# Autodesk Inventor assembly: Cube 1x1 V5
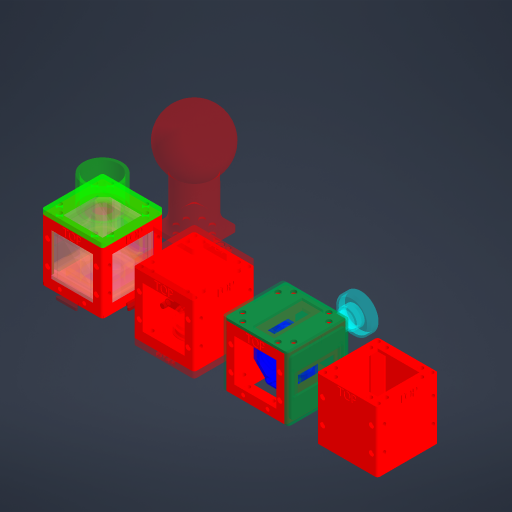
[picture p0: Inventor's stored thumbnail of the model, 512x512]
Saved by Autodesk Inventor 2023.4 (Build 274418000, 418)
## iProperties
Created: 2022-07-25
Part Number: Cube 1x1 V5
Document SubType Name: Assembly
Designer: xSibe
Author: xSibe
## Documents named in this file (60)
- C:\.Laptop\.Work\Projects\Project Protocube\Protocube\CAD, STL, OBJ Files\1 CAD\Cube 1x1 V5.iam
- C:\.Laptop\.Work\Projects\Project Protocube\Protocube\CAD, STL, OBJ Files\1 CAD\Cubes\Cube 1x1 Bottom V5.ipt
- C:\.Laptop\.Work\Projects\Project Protocube\Protocube\CAD, STL, OBJ Files\1 CAD\Cubes\Cube 1x1 Top V5.ipt
- C:\.Laptop\.Work\Projects\Project Protocube\Protocube\CAD, STL, OBJ Files\1 CAD\Lens\One Inch Lens Mount (V5).ipt
- C:\.Laptop\.Work\Projects\Project Protocube\Protocube\CAD, STL, OBJ Files\1 CAD\Lens\Half Inch Lens Mount (V5).ipt
- C:\.Laptop\.Work\Projects\Project Protocube\Protocube\CAD, STL, OBJ Files\1 CAD\Objective\Objective Mount.ipt
- C:\.Laptop\.Work\Projects\Project Protocube\Protocube\CAD, STL, OBJ Files\1 CAD\Mirror\Mirror Base Vertical.ipt
- C:\.Laptop\.Work\Projects\Project Protocube\Protocube\CAD, STL, OBJ Files\1 CAD\Mirror\Mirror Plate Vertical.ipt
- C:\.Laptop\.Work\Projects\Project Protocube\Protocube\CAD, STL, OBJ Files\1 CAD\Dichroic\Dichroic Mirror Mount.ipt
- C:\.Laptop\.Work\Projects\Project Protocube\Protocube\CAD, STL, OBJ Files\1 CAD\Accessories\Top Mount (SM1).ipt
- C:\.Laptop\.Work\Projects\Project Protocube\Protocube\CAD, STL, OBJ Files\1 CAD\Accessories\Flashlight Mount V1.ipt
- C:\.Laptop\.Work\Projects\Project Protocube\Protocube\CAD, STL, OBJ Files\1 CAD\Camera\Camera Mount Side.ipt
- C:\.Laptop\.Work\Projects\Project Protocube\Protocube\CAD, STL, OBJ Files\1 CAD\Lens\SM1 Lens Mount (V5).ipt
- C:\.Laptop\.Work\Projects\Project Protocube\Protocube\CAD, STL, OBJ Files\1 CAD\Mirror\Mirror Base Horizontal.ipt
- C:\.Laptop\.Work\Projects\Project Protocube\Protocube\CAD, STL, OBJ Files\1 CAD\Mirror\Mirror Plate Horizontal.ipt
- C:\.Laptop\.Work\Projects\Project Protocube\Protocube\CAD, STL, OBJ Files\1 CAD\Tools\Baseplate V5 Press.ipt
- C:\.Laptop\.Work\Projects\Project Protocube\Protocube\CAD, STL, OBJ Files\1 CAD\Tools\Laser Alignment Tool V1.ipt
- C:\.Laptop\.Work\Projects\Project Protocube\Protocube\CAD, STL, OBJ Files\1 CAD\Filter\Filter Mount (SM05).ipt
- C:\.Laptop\.Work\Projects\Project Protocube\Protocube\CAD, STL, OBJ Files\1 CAD\Filter\Filter Mount (SM1).ipt
- C:\.Laptop\.Work\Projects\Project Protocube\Protocube\CAD, STL, OBJ Files\1 CAD\Covers\Inner Cover Side.ipt
- C:\.Laptop\.Work\Projects\Project Protocube\Protocube\CAD, STL, OBJ Files\1 CAD\Covers\Inner Cover Side Open.ipt
- C:\.Laptop\.Work\Projects\Project Protocube\Protocube\CAD, STL, OBJ Files\1 CAD\Cubes\Cube 1x1 Top V5 Closed.ipt
- C:\.Laptop\.Work\Projects\Project Protocube\Protocube\CAD, STL, OBJ Files\1 CAD\Cubes\Cube 1x1 Bottom V5 Closed.ipt
- C:\.Laptop\.Work\Projects\Project Protocube\Protocube\CAD, STL, OBJ Files\1 CAD\Cubes\Cube 1x1 Bottom V5 Closed Slotted.ipt
- C:\.Laptop\.Work\Projects\Project Protocube\Protocube\CAD, STL, OBJ Files\1 CAD\Cubes\Cube 1x1 Top V5 Closed Slotted.ipt
- C:\.Laptop\.Work\Projects\Project Protocube\Protocube\CAD, STL, OBJ Files\1 CAD\Lens\Half Inch Lens Mount Cover (V5).ipt
- C:\.Laptop\.Work\Projects\Project Protocube\Protocube\CAD, STL, OBJ Files\1 CAD\Lens\One Inch Lens Mount Cover (V5).ipt
- C:\.Laptop\.Work\Projects\Project Protocube\Protocube\CAD, STL, OBJ Files\1 CAD\Tools\Laser Alignment Tool V2.ipt
- C:\.Laptop\.Work\Projects\Project Protocube\Protocube\CAD, STL, OBJ Files\1 CAD\Lens\SM05 Lens Mount (V5).ipt
- C:\.Laptop\.Work\Projects\Project Protocube\Protocube\CAD, STL, OBJ Files\1 CAD\Laser\Laser Switch.ipt
- C:\.Laptop\.Work\Projects\Project Protocube\Protocube\CAD, STL, OBJ Files\1 CAD\Laser\Laser Holder (USB Laser).ipt
- C:\.Laptop\.Work\Projects\Project Protocube\Protocube\CAD, STL, OBJ Files\1 CAD\XYZ Stage\Z Stage Body V5.ipt
- C:\.Laptop\.Work\Projects\Project Protocube\Protocube\CAD, STL, OBJ Files\1 CAD\Accessories\Top Mount (SM05).ipt
- C:\.Laptop\.Work\Projects\Project Protocube\Protocube\CAD, STL, OBJ Files\1 CAD\Tools\Cube 1x1 V5 Bot Press.ipt
- C:\.Laptop\.Work\Projects\Project Protocube\Protocube\CAD, STL, OBJ Files\1 CAD\Tools\Cube 1x1 V5 Top Press.ipt
- C:\.Laptop\.Work\Projects\Project Protocube\Protocube\CAD, STL, OBJ Files\1 CAD\Filter\Filter Adapter (SM1).ipt
- C:\.Laptop\.Work\Projects\Project Protocube\Protocube\CAD, STL, OBJ Files\1 CAD\Filter\Filter Adapter (SM05).ipt
- C:\.Laptop\.Work\Projects\Project Protocube\Protocube\CAD, STL, OBJ Files\1 CAD\Laser\Laser Holder (Smaller).ipt
- C:\.Laptop\.Work\Projects\Project Protocube\Protocube\CAD, STL, OBJ Files\1 CAD\Cubes\Cube 1x1 Bottom V5 Closed Vertical.ipt
- C:\.Laptop\.Work\Projects\Project Protocube\Protocube\CAD, STL, OBJ Files\1 CAD\Sample\Sample Holder.ipt
- C:\.Laptop\.Work\Projects\Project Protocube\Protocube\CAD, STL, OBJ Files\1 CAD\Sample\Sample Clamp.ipt
- C:\.Laptop\.Work\Projects\Project Protocube\Protocube\CAD, STL, OBJ Files\1 CAD\Tools\SM1 Press Inner.ipt
- C:\.Laptop\.Work\Projects\Project Protocube\Protocube\CAD, STL, OBJ Files\1 CAD\Tools\SM1 Press Outer.ipt
- C:\.Laptop\.Work\Projects\Project Protocube\Protocube\CAD, STL, OBJ Files\1 CAD\Covers\Outer Cover Open.ipt
- C:\.Laptop\.Work\Projects\Project Protocube\Protocube\CAD, STL, OBJ Files\1 CAD\Baseplates\Interlinking Baseplate.ipt
- C:\.Laptop\.Work\Projects\Project Protocube\Protocube\CAD, STL, OBJ Files\1 CAD\Accessories\Tunnel Vertical.ipt
- C:\.Laptop\.Work\Projects\Project Protocube\Protocube\CAD, STL, OBJ Files\1 CAD\Accessories\Tunnel Horizontal.ipt
- C:\.Laptop\.Work\Projects\Project Protocube\Protocube\CAD, STL, OBJ Files\1 CAD\Baseplates\Interlinking Baseplate Spacer.ipt
- C:\.Laptop\.Work\Projects\Project Protocube\Protocube\CAD, STL, OBJ Files\1 CAD\Baseplates\Interlinking Baseplate Pathed.ipt
- C:\.Laptop\.Work\Projects\Project Protocube\Protocube\CAD, STL, OBJ Files\1 CAD\Baseplates\Interlinking Baseplate Pathed Male.ipt
- C:\.Laptop\.Work\Projects\Project Protocube\Protocube\CAD, STL, OBJ Files\1 CAD\Baseplates\Interlinking Baseplate Pathed Female.ipt
- C:\.Laptop\.Work\Projects\Project Protocube\Protocube\CAD, STL, OBJ Files\1 CAD\Baseplates\Interlinking Baseplate Pathed Angle V2.ipt
- C:\.Laptop\.Work\Projects\Project Protocube\Protocube\CAD, STL, OBJ Files\1 CAD\Baseplates\Interlinking Baseplate Pathed Angle V1.ipt
- C:\.Laptop\.Work\Projects\Project Protocube\Protocube\CAD, STL, OBJ Files\1 CAD\Covers\Outer Cover Top Open.ipt
- C:\.Laptop\.Work\Projects\Project Protocube\Protocube\CAD, STL, OBJ Files\1 CAD\Tools\SM1 Removal Tool.ipt
- C:\.Laptop\.Work\Projects\Project Protocube\Protocube\CAD, STL, OBJ Files\1 CAD\Covers\Outer Cover.ipt
- C:\.Laptop\.Work\Projects\Project Protocube\Protocube\CAD, STL, OBJ Files\1 CAD\Covers\Outer Cover Top.ipt
- C:\.Laptop\.Work\Projects\Project Protocube\Protocube\CAD, STL, OBJ Files\1 CAD\Covers\Outer Cover Full.ipt
- C:\.Laptop\.Work\Projects\Project Protocube\Protocube\CAD, STL, OBJ Files\1 CAD\Covers\Outer Cover Side Open.ipt
- C:\.Laptop\.Work\Projects\Project Protocube\Protocube\CAD, STL, OBJ Files\1 CAD\Covers\Outer Cover Side.ipt
## Components (60 placed, 59 different names)
1. Cube 1x1 Top V5:1 — Mate:1, Mate:2, Mate:3, Mate:4, Mate:5, Mate:6, Mate:40, Flush:23, Flush:24, Mate:60, Mate:61, Mate:62, Mate:63, Mate:64, Mate:65, Flush:39
2. Cube 1x1 Bottom V5:1 — Mate:1, Mate:2, Mate:3, Mate:39, Flush:21, Mate:70, Mate:85, Flush:35, Flush:36, Mate:86, Flush:37
3. Cube 1x1 Top V5 Closed:1 — Mate:40, Flush:23, Flush:24, Mate:41, Mate:42, Mate:43, Mate:77, Mate:78, Mate:79
4. Cube 1x1 Bottom V5 Closed:1 — Mate:41, Mate:42, Mate:43, Mate:54, Mate:55, Mate:56, Mate:76, Mate:80, Mate:81, Mate:82, Mate:83, Flush:30, Mate:75
5. Cube 1x1 Top V5 Closed Slotted:1 — Mate:51, Mate:52, Mate:53
6. Cube 1x1 Bottom V5 Closed Slotted:1 — Mate:51, Mate:52, Mate:53, Mate:54, Mate:55, Mate:56, Mate:66, Flush:25, Flush:26, Flush:32, Flush:33, Flush:34, Flush:42
7. Cube 1x1 Top V5:2 — Mate:67, Mate:68, Mate:69
8. Cube 1x1 Bottom V5 Closed Vertical:1 — Mate:66, Flush:25, Flush:26, Mate:67, Mate:68, Mate:69
9. Laser Alignment Tool V1:1 — Flush:18
10. Laser Alignment Tool V2:1
11. Baseplate V5 Press:1 — Flush:15
12. Cube 1x1 V5 Bot Press:1 — Mate:76, Mate:80, Mate:81
13. Cube 1x1 V5 Top Press:1 — Mate:77, Mate:78, Mate:79
14. SM1 Removal Tool:1 — Mate:87, Flush:40, Flush:41
15. SM1 Press Outer:1 — Flush:29, Mate:74, Mate:75, Flush:40, Flush:41
16. SM1 Press Inner:1 — Flush:29, Mate:74, Mate:87
17. Laser Switch:1 — Mate:82, Mate:83, Flush:30
18. Z Stage Body V5:1
19. Half Inch Lens Mount Cover (V5):1
20. One Inch Lens Mount Cover (V5):1
21. Half Inch Lens Mount (V5):1
22. One Inch Lens Mount (V5):1 — Flush:1
23. SM05 Lens Mount (V5):1
24. SM1 Lens Mount (V5):1
25. Filter Mount (SM05):1 — Flush:19
26. Filter Mount (SM1):1
27. Laser Holder (USB Laser):1
28. Laser Holder (Smaller):1
29. Mirror Base Vertical:1 — Flush:5
30. Mirror Plate Vertical:1
31. Mirror Base Horizontal:1 — Flush:12, Flush:14
32. Mirror Plate Horizontal:1 — Mate:38, Flush:13, Flush:14
33. Dichroic Mirror Mount:1 — Flush:6
34. Camera Mount Side:1 — Flush:7
35. Objective Mount:1 — Flush:4
36. Tunnel Horizontal:1 — Mate:86, Flush:37, Flush:39
37. Tunnel Vertical:1 — Mate:85, Flush:35, Flush:36
38. Sample Holder:1 — Mate:70, Mate:71, Flush:27, Mate:72
39. Sample Clamp:1 — Mate:72, Mate:73, Flush:28
40. Interlinking Baseplate:1
41. Interlinking Baseplate Spacer:1
42. Interlinking Baseplate Pathed:1
43. Interlinking Baseplate Pathed Male:1
44. Interlinking Baseplate Pathed Female:1
45. Interlinking Baseplate Pathed Angle V2:1
46. Interlinking Baseplate Pathed Angle V1:1
47. Filter Adapter (SM1):1 — Mate:84, Flush:31, Flush:32, Flush:33, Flush:34
48. Filter Adapter (SM05):1 — Mate:84, Flush:31
49. Top Mount (SM1):1 — Mate:4, Mate:5, Mate:6
50. Top Mount (SM05):1 — Mate:60, Mate:61, Mate:62
51. Flashlight Mount V1:1 — Mate:63, Mate:64, Mate:65
52. Outer Cover Side Open:1 — Flush:42, Flush:43
53. Outer Cover Side:1 — Flush:43
54. Outer Cover Top Open:1
55. Outer Cover Top:1
56. Outer Cover Open:1
57. Outer Cover:1
58. Outer Cover Full:1
59. Inner Cover Side:1 — Flush:20, Mate:39, Flush:21
60. Inner Cover Side Open:1
## Relationships (79: Mate 46, Flush 33)
- Mate:1: Cube 1x1 Top V5:1 ↔ Cube 1x1 Bottom V5:1
- Mate:2: Cube 1x1 Top V5:1 ↔ Cube 1x1 Bottom V5:1
- Mate:3: Cube 1x1 Top V5:1 ↔ Cube 1x1 Bottom V5:1
- Flush:1: One Inch Lens Mount (V5):1
- Flush:4: Objective Mount:1
- Flush:5: Mirror Base Vertical:1
- Flush:6: Dichroic Mirror Mount:1
- Mate:4: Cube 1x1 Top V5:1 ↔ Top Mount (SM1):1
- Mate:5: Cube 1x1 Top V5:1 ↔ Top Mount (SM1):1
- Mate:6: Cube 1x1 Top V5:1 ↔ Top Mount (SM1):1
- Flush:7: Camera Mount Side:1
- Flush:12: Mirror Base Horizontal:1
- Mate:38: Mirror Plate Horizontal:1
- Flush:13: Mirror Plate Horizontal:1
- Flush:14: Mirror Base Horizontal:1 ↔ Mirror Plate Horizontal:1
- Flush:15: Baseplate V5 Press:1
- Flush:18: Laser Alignment Tool V1:1
- Flush:19: Filter Mount (SM05):1
- Flush:20: Inner Cover Side:1
- Mate:39: Cube 1x1 Bottom V5:1 ↔ Inner Cover Side:1
- Flush:21: Cube 1x1 Bottom V5:1 ↔ Inner Cover Side:1
- Mate:40 (25 mm): Cube 1x1 Top V5:1 ↔ Cube 1x1 Top V5 Closed:1
- Flush:23: Cube 1x1 Top V5:1 ↔ Cube 1x1 Top V5 Closed:1
- Flush:24: Cube 1x1 Top V5:1 ↔ Cube 1x1 Top V5 Closed:1
- Mate:41: Cube 1x1 Top V5 Closed:1 ↔ Cube 1x1 Bottom V5 Closed:1
- Mate:42: Cube 1x1 Top V5 Closed:1 ↔ Cube 1x1 Bottom V5 Closed:1
- Mate:43: Cube 1x1 Top V5 Closed:1 ↔ Cube 1x1 Bottom V5 Closed:1
- Mate:51: Cube 1x1 Top V5 Closed Slotted:1 ↔ Cube 1x1 Bottom V5 Closed Slotted:1
- Mate:52: Cube 1x1 Top V5 Closed Slotted:1 ↔ Cube 1x1 Bottom V5 Closed Slotted:1
- Mate:53: Cube 1x1 Top V5 Closed Slotted:1 ↔ Cube 1x1 Bottom V5 Closed Slotted:1
- Mate:54 (25 mm): Cube 1x1 Bottom V5 Closed:1 ↔ Cube 1x1 Bottom V5 Closed Slotted:1
- Mate:55: Cube 1x1 Bottom V5 Closed:1 ↔ Cube 1x1 Bottom V5 Closed Slotted:1
- Mate:56: Cube 1x1 Bottom V5 Closed:1 ↔ Cube 1x1 Bottom V5 Closed Slotted:1
- Mate:60: Cube 1x1 Top V5:1 ↔ Top Mount (SM05):1
- Mate:61: Cube 1x1 Top V5:1 ↔ Top Mount (SM05):1
- Mate:62: Cube 1x1 Top V5:1 ↔ Top Mount (SM05):1
- Mate:63: Cube 1x1 Top V5:1 ↔ Flashlight Mount V1:1
- Mate:64: Cube 1x1 Top V5:1 ↔ Flashlight Mount V1:1
- Mate:65: Cube 1x1 Top V5:1 ↔ Flashlight Mount V1:1
- Mate:66 (25 mm): Cube 1x1 Bottom V5 Closed Slotted:1 ↔ Cube 1x1 Bottom V5 Closed Vertical:1
- Flush:25: Cube 1x1 Bottom V5 Closed Slotted:1 ↔ Cube 1x1 Bottom V5 Closed Vertical:1
- Flush:26: Cube 1x1 Bottom V5 Closed Slotted:1 ↔ Cube 1x1 Bottom V5 Closed Vertical:1
- Mate:67: Cube 1x1 Top V5:2 ↔ Cube 1x1 Bottom V5 Closed Vertical:1
- Mate:68: Cube 1x1 Top V5:2 ↔ Cube 1x1 Bottom V5 Closed Vertical:1
- Mate:69: Cube 1x1 Top V5:2 ↔ Cube 1x1 Bottom V5 Closed Vertical:1
- Mate:70: Cube 1x1 Bottom V5:1 ↔ Sample Holder:1
- Mate:71: Sample Holder:1
- Flush:27: Sample Holder:1
- Mate:72: Sample Holder:1 ↔ Sample Clamp:1
- Mate:73: Sample Clamp:1
- Flush:28: Sample Clamp:1
- Flush:29: SM1 Press Outer:1 ↔ SM1 Press Inner:1
- Mate:74: SM1 Press Outer:1 ↔ SM1 Press Inner:1
- Mate:75: Cube 1x1 Bottom V5 Closed:1 ↔ SM1 Press Outer:1
- Mate:76: Cube 1x1 Bottom V5 Closed:1 ↔ Cube 1x1 V5 Bot Press:1
- Mate:77: Cube 1x1 Top V5 Closed:1 ↔ Cube 1x1 V5 Top Press:1
- Mate:78: Cube 1x1 Top V5 Closed:1 ↔ Cube 1x1 V5 Top Press:1
- Mate:79: Cube 1x1 Top V5 Closed:1 ↔ Cube 1x1 V5 Top Press:1
- Mate:80: Cube 1x1 Bottom V5 Closed:1 ↔ Cube 1x1 V5 Bot Press:1
- Mate:81: Cube 1x1 Bottom V5 Closed:1 ↔ Cube 1x1 V5 Bot Press:1
- Mate:82: Cube 1x1 Bottom V5 Closed:1 ↔ Laser Switch:1
- Mate:83: Cube 1x1 Bottom V5 Closed:1 ↔ Laser Switch:1
- Flush:30 (-25 mm): Cube 1x1 Bottom V5 Closed:1 ↔ Laser Switch:1
- Mate:84: Filter Adapter (SM1):1 ↔ Filter Adapter (SM05):1
- Flush:31: Filter Adapter (SM1):1 ↔ Filter Adapter (SM05):1
- Flush:32: Cube 1x1 Bottom V5 Closed Slotted:1 ↔ Filter Adapter (SM1):1
- Flush:33 (50 mm): Cube 1x1 Bottom V5 Closed Slotted:1 ↔ Filter Adapter (SM1):1
- Flush:34 (-25 mm): Cube 1x1 Bottom V5 Closed Slotted:1 ↔ Filter Adapter (SM1):1
- Mate:85: Cube 1x1 Bottom V5:1 ↔ Tunnel Vertical:1
- Flush:35 (0.075 mm): Cube 1x1 Bottom V5:1 ↔ Tunnel Vertical:1
- Flush:36 (0.075 mm): Cube 1x1 Bottom V5:1 ↔ Tunnel Vertical:1
- Mate:86: Cube 1x1 Bottom V5:1 ↔ Tunnel Horizontal:1
- Flush:37 (0.075 mm): Cube 1x1 Bottom V5:1 ↔ Tunnel Horizontal:1
- Flush:39 (0.075 mm): Cube 1x1 Top V5:1 ↔ Tunnel Horizontal:1
- Mate:87: SM1 Removal Tool:1 ↔ SM1 Press Inner:1
- Flush:40: SM1 Removal Tool:1 ↔ SM1 Press Outer:1
- Flush:41: SM1 Removal Tool:1 ↔ SM1 Press Outer:1
- Flush:42: Cube 1x1 Bottom V5 Closed Slotted:1 ↔ Outer Cover Side Open:1
- Flush:43: Outer Cover Side Open:1 ↔ Outer Cover Side:1
